# Autodesk Inventor assembly: ASDSAttachmentAssemblyUpdated
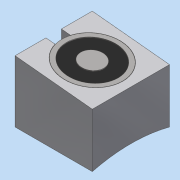
[picture p0: Inventor's stored thumbnail of the model, 180x180]
Saved by Autodesk Inventor 2017.3 (Build 213256000, 256)
## iProperties
Created: 2018-08-31
Part Number: ASDSAttachmentAssemblyUpdated
Document SubType Name: Assembly
Designer: Derek Wider
Author: Derek Wider
## Documents named in this file (4)
- G:\Projects\Submarine\Submarine-project\CAD\midships\ASDSAttachment\ASDSAttachmentAssemblyUpdated.iam
- G:\Projects\Submarine\Submarine-project\CAD\midships\ASDSAttachment\electromagnetHolder.ipt
- G:\Projects\Submarine\Submarine-project\CAD\midships\ASDSAttachment\electromagnet.ipt
- G:\Projects\Submarine\Submarine-project\CAD\common\ThreadedRod_Nuts_Bolts\Bolt_FlatHead_Phillips_Thread_M3_5mm.ipt
## Components (3 placed, 3 different names)
1. electromagnetHolder:1 — Mate:1, Mate:2
2. electromagnet:1 — Mate:1, Mate:2, Mate:3, Flush:1
3. Bolt_FlatHead_Phillips_Thread_M3_5mm:1 — Mate:3, Flush:1
## Relationships (4: Mate 3, Flush 1)
- Mate:1: electromagnetHolder:1 ↔ electromagnet:1
- Mate:2: electromagnetHolder:1 ↔ electromagnet:1
- Mate:3: electromagnet:1 ↔ Bolt_FlatHead_Phillips_Thread_M3_5mm:1
- Flush:1 (-1.27 mm): electromagnet:1 ↔ Bolt_FlatHead_Phillips_Thread_M3_5mm:1
